# Autodesk Inventor assembly: Potencia
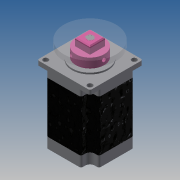
[picture p0: Inventor's stored thumbnail of the model, 180x180]
Saved by Autodesk Inventor 2017 (Build 210142000, 142)
## iProperties
Part Number: Potencia
Material: Genérico
Document SubType Name: Assembly
Designer: FABLAB
Author: FABLAB
## Documents named in this file (3)
- C:\Users\FABLAB\Dropbox\E\Caja Motriz\transmision Engranajes\Potencia.iam
- C:\Users\FABLAB\Dropbox\E\Caja Motriz\Piezas\Motor.ipt
- C:\Users\FABLAB\Dropbox\E\Caja Motriz\transmision Engranajes\Polea Compuesta.iam
## Components (2 placed, 2 different names)
1. Motor:1 — Insertar:1
2. Polea Compuesta:1 [sub-assembly] — Insertar:1
## Relationships (1: Insert 1)
- Insertar:1: Motor:1 ↔ Polea Compuesta:1
